# Autodesk Inventor assembly: PIHTI-for-Boron_1
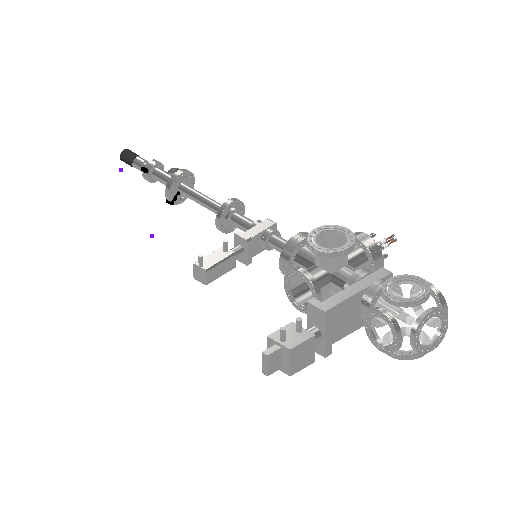
[picture p0: Inventor's stored thumbnail of the model, 512x512]
Saved by Autodesk Inventor 2026.2 (Build 302298000, 298)
## iProperties
Created: 2024-05-09
Part Number: PIHTI-for-Boron_1
Document SubType Name: Assembly
Designer: kuzmin
Mass: 19614.5 g
Surface Area: 13609.5 cm^2
Volume: 3689.47 cm^3
Density: 5.31636 g/cm^3
Author: kuzmin
## Documents named in this file (17)
- D:\repos\PIHTI\Plasma Vessel_1\PIHTI-for-boron_1\PIHTI-for-Boron_1.iam
- D:\repos\PIHTI\Plasma Vessel\Plasma-vacuum-cross\Plasma-vacuum-vessel-152IC-cross.iam
- D:\repos\PIHTI\Plasma Vessel\Plasma-Box\Plasma-box-hayashi-aka-upgrade.iam
- D:\repos\PIHTI\ContentCenter\Fastners\M3x8-SHCS.ipt
- D:\repos\PIHTI\Plasma Vessel\Plasma-Box\probe-gate-with-spindel.iam
- D:\repos\PIHTI\Plasma Vessel\Cathode-Anode-Flange\cf70_spacer.ipt
- D:\repos\PIHTI\Plasma Vessel\entrance-mesh-assembly.iam
- D:\repos\PIHTI\Plasma Vessel\probe-port-mesh-welded.iam
- D:\repos\PIHTI\ContentCenter\CF-parts\CF-Flanges\CF_152-70.ipt
- D:\repos\PIHTI\ContentCenter\CF-parts\CF70-nipple\CF70-nipple.iam
- D:\repos\PIHTI\ContentCenter\CF-parts\CF70-gate-valve\Gatevalve_70_pneumatic.iam
- D:\repos\PIHTI\Plasma Vessel_1\PIHTI-for-boron_1\parts\gate_valve\gate_valve_assembly.iam
- D:\repos\PIHTI\Plasma Vessel_1\PIHTI-for-boron_1\parts\contents\CF_114-70.ipt
- D:\repos\PIHTI\BoronProbe_5\BoronProbe_5.iam
- D:\repos\PIHTI\Plasma Vessel_1\PIHTI-for-boron_1\parts\Cathode-Anode-Flange\Cathode-Anode-70IC-flange-with-feeds.iam
- D:\repos\PIHTI\Plasma Vessel_1\PIHTI-for-boron_1\parts\Plasma-Flange-2024\cathode-box-on-a-flange.iam
- D:\repos\PIHTI\Plasma Vessel_1\PIHTI-for-boron_1\parts\Plasma-vacuum-vessel\Plasma-vacuum-vessel-152IC-cross-L205p8.iam
## Components (24 placed, 16 different names)
1. Plasma-vacuum-vessel-152IC-cross:1 [sub-assembly] — メイト:1, フラッシュ:1, フラッシュ:2, リジッド:18, メイト:22, メイト:23, メイト:24, メイト:34, メイト:35, メイト:36
2. Plasma-box-hayashi-aka-upgrade:1 [sub-assembly] — メイト:3, メイト:4, Hinge Angle, メイト:13, メイト:17
3. probe-gate-with-spindel:1 [sub-assembly] — メイト:3, メイト:4, Hinge Angle
4. cf70_spacer:1 — メイト:37, メイト:39, メイト:40, メイト:41, メイト:42, メイト:43
5. entrance-mesh-assembly:1 [sub-assembly] — メイト:13, メイト:17, メイト:19
6. probe-port-mesh-welded:1 [sub-assembly] — メイト:19
7. CF_152-70:1 — リジッド:18, リジッド:21
8. CF70-nipple:1 [sub-assembly] — リジッド:21, リジッド:22, メイト:31
9. CF70-nipple:2 [sub-assembly] — リジッド:23, メイト:29, メイト:31, メイト:32
10. Gatevalve_70_pneumatic:1 [sub-assembly] — リジッド:22, リジッド:23
11. gate_valve_assembly:1 [sub-assembly] — メイト:22, メイト:23, メイト:24, メイト:44, メイト:45, メイト:46
12. CF_114-70:1 — メイト:29, メイト:32, メイト:33, メイト:47
13. BoronProbe_5:1 [sub-assembly] — メイト:33, メイト:47
14. cathode-box-on-a-flange:1 [sub-assembly] — メイト:34, メイト:35, メイト:36, メイト:37, メイト:39, メイト:40
15. Cathode-Anode-70IC-flange-with-feeds:1 [sub-assembly] — メイト:41, メイト:42, メイト:43
16. Plasma-vacuum-vessel-152IC-cross-L205p8:1 [sub-assembly] — メイト:44, メイト:45, メイト:46
17. SS ISO 4762 M3 x 8:5
18. SS ISO 4762 M3 x 8:6
19. SS ISO 4762 M3 x 8:7
20. SS ISO 4762 M3 x 8:8
21. SS ISO 4762 M3 x 8:1
22. SS ISO 4762 M3 x 8:2
23. SS ISO 4762 M3 x 8:3
24. SS ISO 4762 M3 x 8:4
## Relationships (33: Mate 26, WeldJoint 4, Flush 2, Angle 1)
- メイト:1 [Mate]: Plasma-vacuum-vessel-152IC-cross:1
- フラッシュ:1 [Flush]: Plasma-vacuum-vessel-152IC-cross:1
- フラッシュ:2 [Flush]: Plasma-vacuum-vessel-152IC-cross:1
- メイト:3 [Mate]: Plasma-box-hayashi-aka-upgrade:1 ↔ probe-gate-with-spindel:1
- メイト:4 [Mate]: Plasma-box-hayashi-aka-upgrade:1 ↔ probe-gate-with-spindel:1
- Hinge Angle [Angle] (45 deg): Plasma-box-hayashi-aka-upgrade:1 ↔ probe-gate-with-spindel:1
- メイト:13 [Mate]: Plasma-box-hayashi-aka-upgrade:1 ↔ entrance-mesh-assembly:1
- メイト:17 [Mate]: Plasma-box-hayashi-aka-upgrade:1 ↔ entrance-mesh-assembly:1
- メイト:19 [Mate]: entrance-mesh-assembly:1 ↔ probe-port-mesh-welded:1
- リジッド:18 [WeldJoint]: Plasma-vacuum-vessel-152IC-cross:1 ↔ CF_152-70:1
- リジッド:21 [WeldJoint]: CF_152-70:1 ↔ CF70-nipple:1
- リジッド:22 [WeldJoint]: CF70-nipple:1 ↔ Gatevalve_70_pneumatic:1
- リジッド:23 [WeldJoint]: CF70-nipple:2 ↔ Gatevalve_70_pneumatic:1
- メイト:22 [Mate]: Plasma-vacuum-vessel-152IC-cross:1 ↔ gate_valve_assembly:1
- メイト:23 [Mate]: Plasma-vacuum-vessel-152IC-cross:1 ↔ gate_valve_assembly:1
- メイト:24 [Mate]: Plasma-vacuum-vessel-152IC-cross:1 ↔ gate_valve_assembly:1
- メイト:29 [Mate]: CF70-nipple:2 ↔ CF_114-70:1
- メイト:31 [Mate]: CF70-nipple:1 ↔ CF70-nipple:2
- メイト:32 [Mate]: CF70-nipple:2 ↔ CF_114-70:1
- メイト:33 [Mate]: CF_114-70:1 ↔ BoronProbe_5:1
- メイト:34 [Mate]: Plasma-vacuum-vessel-152IC-cross:1 ↔ cathode-box-on-a-flange:1
- メイト:35 [Mate]: Plasma-vacuum-vessel-152IC-cross:1 ↔ cathode-box-on-a-flange:1
- メイト:36 [Mate]: Plasma-vacuum-vessel-152IC-cross:1 ↔ cathode-box-on-a-flange:1
- メイト:37 [Mate]: cf70_spacer:1 ↔ cathode-box-on-a-flange:1
- メイト:39 [Mate]: cf70_spacer:1 ↔ cathode-box-on-a-flange:1
- メイト:40 [Mate]: cf70_spacer:1 ↔ cathode-box-on-a-flange:1
- メイト:41 [Mate]: cf70_spacer:1 ↔ Cathode-Anode-70IC-flange-with-feeds:1
- メイト:42 [Mate]: cf70_spacer:1 ↔ Cathode-Anode-70IC-flange-with-feeds:1
- メイト:43 [Mate]: cf70_spacer:1 ↔ Cathode-Anode-70IC-flange-with-feeds:1
- メイト:44 [Mate]: gate_valve_assembly:1 ↔ Plasma-vacuum-vessel-152IC-cross-L205p8:1
- メイト:45 [Mate]: gate_valve_assembly:1 ↔ Plasma-vacuum-vessel-152IC-cross-L205p8:1
- メイト:46 [Mate]: gate_valve_assembly:1 ↔ Plasma-vacuum-vessel-152IC-cross-L205p8:1
- メイト:47 [Mate]: CF_114-70:1 ↔ BoronProbe_5:1
